# Autodesk Inventor assembly: Assembly1nwe
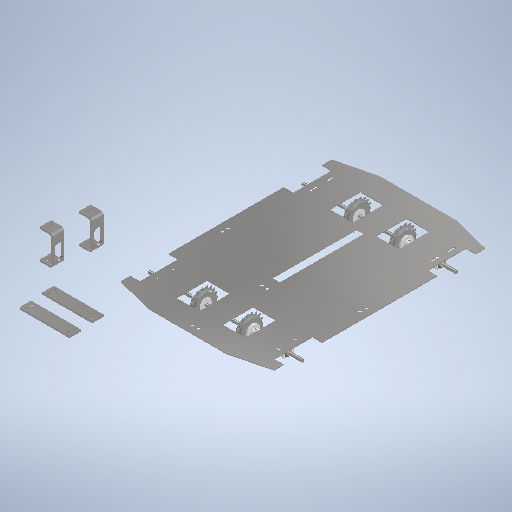
[picture p0: Inventor's stored thumbnail of the model, 512x512]
Saved by Autodesk Inventor 2026.1 (Build 301233020, 233B)
## iProperties
Created: 2026-01-25
Part Number: Assembly1nwe
Document SubType Name: Assembly
Designer: user
Author: user
## Documents named in this file (6)
- D:\asu\machine element design\project\design - Copy\Assembly1nwe.iam
- D:\asu\machine element design\project\design - Copy\chassis.ipt
- D:\asu\machine element design\project\design - Copy\pillow-block-bearing-p08-1.snapshot.17\Pillow Block P08\Pillow Block P08\Pillow Block P08.ipt
- D:\asu\machine element design\project\design - Copy\Assembly shaft 1 sprocect.iam
- D:\asu\machine element design\project\design - Copy\piston bracke11t.ipt
- D:\asu\machine element design\project\design - Copy\up bracket.ipt
## Components (11 placed, 5 different names)
1. chassis:1 — Mate:1, Mate:2, Mate:3, Mate:4, Mate:5, Mate:6, Mate:7, Mate:8, Mate:9, Mate:10, Mate:11, Mate:12, Mate:14, Mate:16
2. Pillow Block P08:1 — Mate:4, Mate:11, Mate:12
3. Pillow Block P08:2 — Mate:2, Mate:5, Mate:6
4. Pillow Block P08:3 — Mate:3, Mate:9, Mate:10, Mate:15
5. Pillow Block P08:4 — Mate:1, Mate:7, Mate:8, Mate:13
6. Assembly shaft 1 sprocect:1 [sub-assembly] — Mate:13, Mate:14
7. Assembly shaft 1 sprocect:2 [sub-assembly] — Mate:15, Mate:16
8. piston bracke11t:1
9. piston bracke11t:2
10. up bracket:1
11. up bracket:2
## Relationships (16: Mate 16)
- Mate:1: chassis:1 ↔ Pillow Block P08:4
- Mate:2: chassis:1 ↔ Pillow Block P08:2
- Mate:3: chassis:1 ↔ Pillow Block P08:3
- Mate:4: chassis:1 ↔ Pillow Block P08:1
- Mate:5: chassis:1 ↔ Pillow Block P08:2
- Mate:6: chassis:1 ↔ Pillow Block P08:2
- Mate:7: chassis:1 ↔ Pillow Block P08:4
- Mate:8: chassis:1 ↔ Pillow Block P08:4
- Mate:9: chassis:1 ↔ Pillow Block P08:3
- Mate:10: chassis:1 ↔ Pillow Block P08:3
- Mate:11: chassis:1 ↔ Pillow Block P08:1
- Mate:12: chassis:1 ↔ Pillow Block P08:1
- Mate:13: Pillow Block P08:4 ↔ Assembly shaft 1 sprocect:1
- Mate:14: chassis:1 ↔ Assembly shaft 1 sprocect:1
- Mate:15: Pillow Block P08:3 ↔ Assembly shaft 1 sprocect:2
- Mate:16: chassis:1 ↔ Assembly shaft 1 sprocect:2
